# Autodesk Inventor assembly: LilypadV5
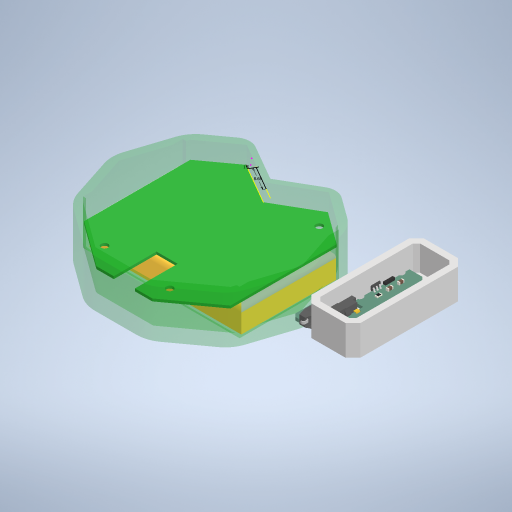
[picture p0: Inventor's stored thumbnail of the model, 512x512]
Saved by Autodesk Inventor 2024 (Build 280153000, 153)
## iProperties
Created: 2023-11-09
Part Number: LilypadV5
Document SubType Name: Assembly
Designer: jevan
Author: jevan
## Documents named in this file (6)
- C:\Users\jevan\Documents\LilypadVR\V5\CAD\Models\LilypadV5.iam
- C:\Users\jevan\Documents\LilypadVR\V5\CAD\Models\ShellMockup_01.ipt
- C:\Users\jevan\Documents\LilypadVR\V5\CAD\Models\Battery.ipt
- C:\Users\jevan\Documents\LilypadVR\V5\CAD\Models\PCB.ipt
- C:\Users\jevan\Documents\LilypadVR\V5\PCB\V5Cattail\V5Cattail\V5Cattail.ipt
- C:\Users\jevan\Documents\LilypadVR\V5\CAD\Sketches\CattailShellMockup_01.ipt
## Components (5 placed, 5 different names)
1. ShellMockup_01:1 — Mate:3, Mate:4, Mate:5, Mate:6, Mate:10
2. Battery:1 — Flush:2, Mate:3, Mate:4, Mate:10
3. PCB:1 — Flush:2, Mate:5, Mate:6
4. V5Cattail:1 — Mate:11
5. CattailShellMockup_01:1 — Mate:11
## Relationships (7: Mate 6, Flush 1)
- Flush:2: Battery:1 ↔ PCB:1
- Mate:3 (0.75 mm): ShellMockup_01:1 ↔ Battery:1
- Mate:4 (1.3 mm): ShellMockup_01:1 ↔ Battery:1
- Mate:5 (0.25 mm): ShellMockup_01:1 ↔ PCB:1
- Mate:6 (0.25 mm): ShellMockup_01:1 ↔ PCB:1
- Mate:10: ShellMockup_01:1 ↔ Battery:1
- Mate:11 (0.5 mm): V5Cattail:1 ↔ CattailShellMockup_01:1
